# Autodesk Inventor assembly: Optical Endstop
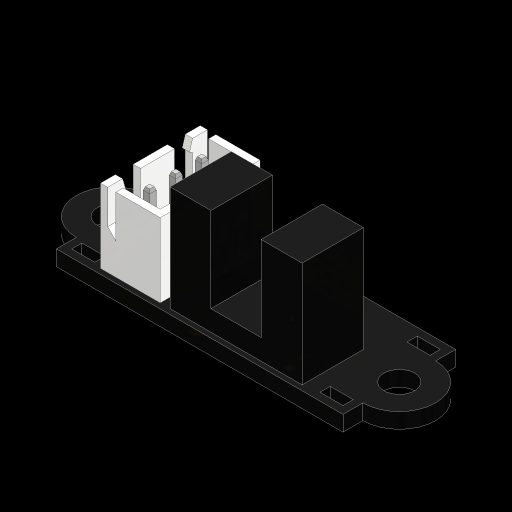
[picture p0: Inventor's stored thumbnail of the model, 512x512]
Saved by Autodesk Inventor 2023 (Build 270158000, 158)
## iProperties
Created: 2023-08-04
Part Number: Optical Endstop
Document SubType Name: Assembly
Designer: tandu
Author: tandu
## iProperties of the stored document OpticalEndstop.ipt
Created: 2023-08-04
Part Number: OpticalEndstop
Material: Generic
Document SubType Name: Modeling
Designer: tandu
Density: 1 g/cm^3
Appearance: Default
Author: tandu
Revision Number: ANY
## iProperties of the stored document OpticalEndstop.iam
Created: 2020-05-16
Part Number: OpticalEndstop
Description: STEP AP214
Document SubType Name: Assembly
Designer: tandu
Sending System: SolidWorks 2019
Preprocessor: SwSTEP 2.0
Title: OpticalEndstop.STEP
Revision Number: ANY
## iProperties of the stored document JST - XH - Thru (V) - 3Pin - 2.54mm.stp.ipt
Created: 2023-08-04
Part Number: JST - XH - Thru (V) - 3Pin - 2.54mm.stp
Material: Generic
Document SubType Name: Modeling
Designer: tandu
Density: 1 g/cm^3
Appearance: Default
Author: tandu
Revision Number: ANY
## Documents named in this file (6)
- C:\Users\tandu\Documents\GrabCAD\Robotic Arm Project\IndustrialStyledVersion\V1\Optical Endstop.iam
- **C:\Users\tandu\Documents\GrabCAD\Robotic Arm Project\IndustrialStyledVersion\V1\Optical Endstop.iam*LocalDocs*xAaaaa3daAaaaaaaaAaaaabq0Ia*OpticalEndstop.iam
- **C:\Users\tandu\Documents\GrabCAD\Robotic Arm Project\IndustrialStyledVersion\V1\Optical Endstop.iam*LocalDocs*xAaaaawdaAaaaaaaaAaaaakctIe*OpticalEndstop.ipt
- **C:\Users\tandu\Documents\GrabCAD\Robotic Arm Project\IndustrialStyledVersion\V1\Optical Endstop.iam*LocalDocs*xAaaaqvdaAaaaaaaaAaaaabtr4f*JST - XH - Thru (V) - 3Pin - 2.54mm.stp.ipt
- JST - XH - Thru (V) - 3Pin - 2.54mm.stp
- C:\Users\tandu\Documents\GrabCAD\Robotic Arm Project\IndustrialStyledVersion\V1\References\OpticalEndstop.STEP
## Components (1 placed, 1 different names)
1. OpticalEndstop:1 [sub-assembly] — Mate:1, Mate:2, Mate:3, Mate:4, Mate:5, Mate:6
## Relationships (6: Mate 6)
- Mate:1: OpticalEndstop:1
- Mate:2: OpticalEndstop:1
- Mate:3: OpticalEndstop:1
- Mate:4: OpticalEndstop:1
- Mate:5: OpticalEndstop:1
- Mate:6: OpticalEndstop:1
